# Autodesk Inventor assembly: full assembly
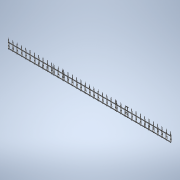
[picture p0: Inventor's stored thumbnail of the model, 180x180]
Saved by Autodesk Inventor 2021 (Build 250183000, 183)
## iProperties
Created: 2021-03-09
Part Number: full assembly
Document SubType Name: Assembly
Designer: Ferdinand Hubbard
Author: Ferdinand Hubbard
## Documents named in this file (7)
- C:\Users\Ferdinand Hubbard\Desktop\solarplane\cad\full assembly.iam
- C:\Users\Ferdinand Hubbard\Desktop\solarplane\cad\centre wing.iam
- C:\Users\Ferdinand Hubbard\Desktop\solarplane\cad\right wing\right wing short.iam
- C:\Users\Ferdinand Hubbard\Desktop\solarplane\cad\right wing\right wing long.iam
- C:\Users\Ferdinand Hubbard\Desktop\solarplane\cad\left wing\left wing short.iam
- C:\Users\Ferdinand Hubbard\Desktop\solarplane\cad\left wing\left wing long.iam
- C:\Users\Ferdinand Hubbard\Desktop\solarplane\cad\angle bracket.ipt
## Components (7 placed, 6 different names)
1. centre wing:1 [sub-assembly] — Mate:1, Mate:2, Mate:3, Mate:4, Mate:9, Mate:10, Mate:11, Mate:12
2. right wing short:1 [sub-assembly] — Mate:1, Mate:2, Mate:3, Mate:4, Mate:5, Mate:6
3. right wing long:1 [sub-assembly] — Mate:5, Mate:6
4. left wing short:1 [sub-assembly] — Mate:9, Mate:10, Mate:11, Mate:12, Mate:15, Mate:16
5. left wing long:1 [sub-assembly] — Mate:15, Mate:16
6. angle bracket:1
7. angle bracket:2
## Relationships (12: Mate 12)
- Mate:1: centre wing:1 ↔ right wing short:1
- Mate:2: centre wing:1 ↔ right wing short:1
- Mate:3: centre wing:1 ↔ right wing short:1
- Mate:4: centre wing:1 ↔ right wing short:1
- Mate:5: right wing short:1 ↔ right wing long:1
- Mate:6: right wing short:1 ↔ right wing long:1
- Mate:9: centre wing:1 ↔ left wing short:1
- Mate:10: centre wing:1 ↔ left wing short:1
- Mate:11: centre wing:1 ↔ left wing short:1
- Mate:12: centre wing:1 ↔ left wing short:1
- Mate:15: left wing short:1 ↔ left wing long:1
- Mate:16: left wing short:1 ↔ left wing long:1
